# Autodesk Inventor assembly: gripperAssembly
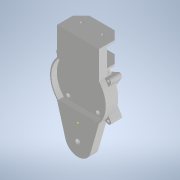
[picture p0: Inventor's stored thumbnail of the model, 180x180]
Saved by Autodesk Inventor 2020 (Build 240168000, 168)
## iProperties
Created: 2019-11-04
Part Number: gripperAssembly
Document SubType Name: Assembly
Designer: kaspe
Author: kaspe
## Documents named in this file (3)
- C:\Users\kaspe\Documents\gripperAssembly.iam
- C:\Users\kaspe\Documents\GripperBase.ipt
- C:\Users\kaspe\Documents\valveMount.ipt
## Components (2 placed, 2 different names)
1. GripperBase:1 — Flush:1
2. valveMount:1 — Flush:1
## Relationships (1: Flush 1)
- Flush:1: GripperBase:1 ↔ valveMount:1
